# Autodesk Inventor assembly: 組合窗_無底
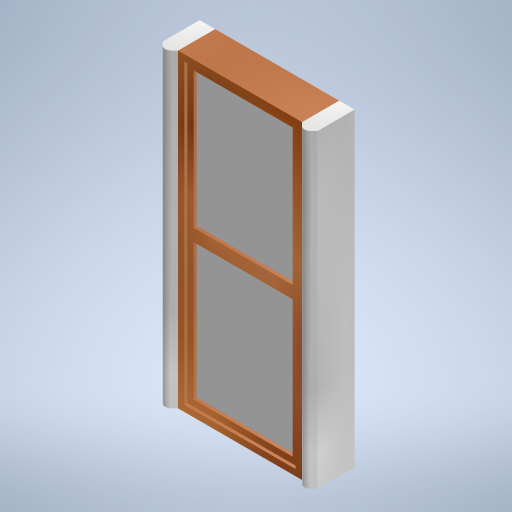
[picture p0: Inventor's stored thumbnail of the model, 512x512]
Saved by Autodesk Inventor 2024.2 (Build 282272000, 272)
## iProperties
Created: 2024-06-03
Part Number: 組合窗_無底
Document SubType Name: Assembly
Designer: User
Author: User
## Documents named in this file (3)
- C:\Users\User\OneDrive - 國立中山大學\桌面\創客基礎\final_project\組合窗_無底.iam
- C:\Users\User\OneDrive - 國立中山大學\桌面\創客基礎\final_project\窗側柱_無底.ipt
- C:\Users\User\OneDrive - 國立中山大學\桌面\創客基礎\final_project\窗_無底.ipt
## Components (3 placed, 2 different names)
1. 窗側柱_無底:1 — 貼合:1, 齊平:1, 齊平:3
2. 窗側柱_無底:2 — 貼合:2, 齊平:2, 齊平:4
3. 窗_無底:1 — 貼合:1, 貼合:2, 齊平:1, 齊平:2, 齊平:3, 齊平:4
## Relationships (6: Flush 4, Mate 2)
- 貼合:1 [Mate]: 窗側柱_無底:1 ↔ 窗_無底:1
- 貼合:2 [Mate]: 窗側柱_無底:2 ↔ 窗_無底:1
- 齊平:1 [Flush]: 窗側柱_無底:1 ↔ 窗_無底:1
- 齊平:2 [Flush]: 窗側柱_無底:2 ↔ 窗_無底:1
- 齊平:3 [Flush]: 窗側柱_無底:1 ↔ 窗_無底:1
- 齊平:4 [Flush]: 窗側柱_無底:2 ↔ 窗_無底:1
